# Autodesk Inventor assembly: PowerDistroAssembly_RevB
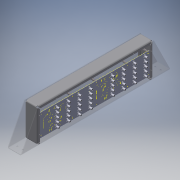
[picture p0: Inventor's stored thumbnail of the model, 180x180]
Saved by Autodesk Inventor 2018 (Build 220112000, 112)
## iProperties
Created: 2018-04-30
Part Number: PowerDistroAssembly_RevB
Document SubType Name: Assembly
Designer: Rich
Author: Rich
## Documents named in this file (6)
- C:\Users\Rich\development\UWaterloo\power-distro.git\SolidModels\PowerDistroAssembly_RevB.iam
- C:\Users\Rich\development\UWaterloo\power-distro.git\SolidModels\Enclosure2_RevB_Outer.ipt
- C:\Users\Rich\development\UWaterloo\power-distro.git\SolidModels\power_distro_pcb_RevB.ipt
- C:\Users\Rich\development\UWaterloo\power-distro.git\SolidModels\rcj-021.iam
- C:\Users\Rich\development\UWaterloo\power-distro.git\SolidModels\Enclosure2_RevB_Inner.ipt
- C:\Users\Rich\development\UWaterloo\power-distro.git\SolidModels\keystone-PN8425.ipt
## Components (53 placed, 5 different names)
1. Enclosure2_RevB_Outer:1 — Flush:1, Flush:2, Mate:1, Mate:4, Mate:5, Mate:6, Mate:7, Mate:8, Mate:9, Mate:10, Mate:11, Mate:12, Mate:13, Mate:14, Mate:15, Mate:16, Mate:17, Mate:18, Mate:19, Mate:20, Mate:21, Mate:22, Mate:23, Mate:24, Mate:25, Mate:26, Mate:27, Mate:28, Mate:29
2. power_distro_pcb_RevB:1 — Mate:2, Angle:1, Tangent:1, Mate:3, Angle:2, Tangent:2, Tangent:3
3. Enclosure2_RevB_Inner:1 — Mate:4, Mate:5, Mate:9
4. keystone-PN8425:1 — Mate:10, Mate:11
5. keystone-PN8425:2 — Mate:15, Mate:27
6. keystone-PN8425:3 — Mate:14, Mate:25
7. keystone-PN8425:4 — Mate:13, Mate:22
8. keystone-PN8425:5 — Mate:12
9. keystone-PN8425:6 — Mate:16, Mate:28
10. keystone-PN8425:7 — Mate:17, Mate:29
11. keystone-PN8425:8 — Mate:18, Mate:20, Mate:26
12. keystone-PN8425:9 — Mate:19, Mate:23
13. keystone-PN8425:10 — Mate:21, Mate:24
14. rcj-021:1 [sub-assembly] — Mate:2, Angle:1, Tangent:1, Mate:6, Mate:7
15. rcj-021:2 [sub-assembly] — Mate:3, Angle:2, Tangent:2, Tangent:3, Mate:8
16. rcj-021:3 [sub-assembly]
17. rcj-021:4 [sub-assembly]
18. rcj-021:5 [sub-assembly]
19. rcj-021:6 [sub-assembly]
20. rcj-021:7 [sub-assembly]
21. rcj-021:8 [sub-assembly]
22. rcj-021:9 [sub-assembly]
23. rcj-021:10 [sub-assembly]
24. rcj-021:11 [sub-assembly]
25. rcj-021:12 [sub-assembly]
26. rcj-021:13 [sub-assembly]
27. rcj-021:14 [sub-assembly]
28. rcj-021:15 [sub-assembly]
29. rcj-021:16 [sub-assembly]
30. rcj-021:17 [sub-assembly]
31. rcj-021:18 [sub-assembly]
32. rcj-021:19 [sub-assembly]
33. rcj-021:20 [sub-assembly]
34. rcj-021:21 [sub-assembly]
35. rcj-021:22 [sub-assembly]
36. rcj-021:23 [sub-assembly]
37. rcj-021:24 [sub-assembly]
38. rcj-021:25 [sub-assembly]
39. rcj-021:26 [sub-assembly]
40. rcj-021:27 [sub-assembly]
41. rcj-021:28 [sub-assembly]
42. rcj-021:29 [sub-assembly]
43. rcj-021:30 [sub-assembly]
44. rcj-021:31 [sub-assembly]
45. rcj-021:32 [sub-assembly]
46. rcj-021:33 [sub-assembly]
47. rcj-021:34 [sub-assembly]
48. rcj-021:35 [sub-assembly]
49. rcj-021:36 [sub-assembly]
50. rcj-021:37 [sub-assembly]
51. rcj-021:38 [sub-assembly]
52. rcj-021:39 [sub-assembly]
53. rcj-021:40 [sub-assembly]
## Component patterns: (20 elements, first: rcj-021:1 + rcj-021:2)
## Relationships (36: Mate 29, Tangent 3, Flush 2, Angle 2)
- Flush:1: Enclosure2_RevB_Outer:1
- Flush:2: Enclosure2_RevB_Outer:1
- Mate:1: Enclosure2_RevB_Outer:1
- Mate:2: power_distro_pcb_RevB:1 ↔ rcj-021:1
- Angle:1 (0 deg): power_distro_pcb_RevB:1 ↔ rcj-021:1
- Tangent:1: power_distro_pcb_RevB:1 ↔ rcj-021:1
- Mate:3: power_distro_pcb_RevB:1 ↔ rcj-021:2
- Angle:2 (0 deg): power_distro_pcb_RevB:1 ↔ rcj-021:2
- Tangent:2: power_distro_pcb_RevB:1 ↔ rcj-021:2
- Tangent:3: power_distro_pcb_RevB:1 ↔ rcj-021:2
- Mate:4: Enclosure2_RevB_Outer:1 ↔ Enclosure2_RevB_Inner:1
- Mate:5: Enclosure2_RevB_Outer:1 ↔ Enclosure2_RevB_Inner:1
- Mate:6: Enclosure2_RevB_Outer:1 ↔ rcj-021:1
- Mate:7: Enclosure2_RevB_Outer:1 ↔ rcj-021:1
- Mate:8: Enclosure2_RevB_Outer:1 ↔ rcj-021:2
- Mate:9: Enclosure2_RevB_Outer:1 ↔ Enclosure2_RevB_Inner:1
- Mate:10: Enclosure2_RevB_Outer:1 ↔ keystone-PN8425:1
- Mate:11: Enclosure2_RevB_Outer:1 ↔ keystone-PN8425:1
- Mate:12: Enclosure2_RevB_Outer:1 ↔ keystone-PN8425:5
- Mate:13: Enclosure2_RevB_Outer:1 ↔ keystone-PN8425:4
- Mate:14: Enclosure2_RevB_Outer:1 ↔ keystone-PN8425:3
- Mate:15: Enclosure2_RevB_Outer:1 ↔ keystone-PN8425:2
- Mate:16: Enclosure2_RevB_Outer:1 ↔ keystone-PN8425:6
- Mate:17: Enclosure2_RevB_Outer:1 ↔ keystone-PN8425:7
- Mate:18: Enclosure2_RevB_Outer:1 ↔ keystone-PN8425:8
- Mate:19: Enclosure2_RevB_Outer:1 ↔ keystone-PN8425:9
- Mate:20: Enclosure2_RevB_Outer:1 ↔ keystone-PN8425:8
- Mate:21: Enclosure2_RevB_Outer:1 ↔ keystone-PN8425:10
- Mate:22: Enclosure2_RevB_Outer:1 ↔ keystone-PN8425:4
- Mate:23: Enclosure2_RevB_Outer:1 ↔ keystone-PN8425:9
- Mate:24: Enclosure2_RevB_Outer:1 ↔ keystone-PN8425:10
- Mate:25: Enclosure2_RevB_Outer:1 ↔ keystone-PN8425:3
- Mate:26: Enclosure2_RevB_Outer:1 ↔ keystone-PN8425:8
- Mate:27: Enclosure2_RevB_Outer:1 ↔ keystone-PN8425:2
- Mate:28: Enclosure2_RevB_Outer:1 ↔ keystone-PN8425:6
- Mate:29: Enclosure2_RevB_Outer:1 ↔ keystone-PN8425:7
